# Autodesk Inventor assembly: SAR340 offset 10 mm
(part 2 of 2)
- to_ball1_7_Z@1 <-> to_rail_Z@10 [Mate]: SAR340-40_r:1 ↔ SAR3_ba:7
- to_ball1_7_YZ@1 <-> to_rail_YZ@10 [Angle] (0 deg): SAR340-40_r:1 ↔ SAR3_ba:7
- to_ball1_8_XY@1 <-> to_rail_XY@11 [Mate]: SAR340-40_r:1 ↔ SAR3_ba:8
- to_ball1_8_Z@1 <-> to_rail_Z@11 [Mate]: SAR340-40_r:1 ↔ SAR3_ba:8
- to_ball1_8_YZ@1 <-> to_rail_YZ@11 [Angle] (0 deg): SAR340-40_r:1 ↔ SAR3_ba:8
- to_ball1_9_XY@1 <-> to_rail_XY@12 [Mate]: SAR340-40_r:1 ↔ SAR3_ba:9
- to_ball1_9_Z@1 <-> to_rail_Z@12 [Mate]: SAR340-40_r:1 ↔ SAR3_ba:9
- to_ball1_9_YZ@1 <-> to_rail_YZ@12 [Angle] (0 deg): SAR340-40_r:1 ↔ SAR3_ba:9
- to_ball1_10_XY@1 <-> to_rail_XY@13 [Mate]: SAR340-40_r:1 ↔ SAR3_ba:10
- to_ball1_10_Z@1 <-> to_rail_Z@13 [Mate]: SAR340-40_r:1 ↔ SAR3_ba:10
- to_ball1_10_YZ@1 <-> to_rail_YZ@13 [Angle] (0 deg): SAR340-40_r:1 ↔ SAR3_ba:10
- to_ball1_11_XY@1 <-> to_rail_XY@14 [Mate]: SAR340-40_r:1 ↔ SAR3_ba:11
- to_ball1_11_Z@1 <-> to_rail_Z@14 [Mate]: SAR340-40_r:1 ↔ SAR3_ba:11
- to_ball1_11_YZ@1 <-> to_rail_YZ@14 [Angle] (0 deg): SAR340-40_r:1 ↔ SAR3_ba:11
- to_ball1_12_XY@1 <-> to_rail_XY@15 [Mate]: SAR340-40_r:1 ↔ SAR3_ba:12
- to_ball1_12_Z@1 <-> to_rail_Z@15 [Mate]: SAR340-40_r:1 ↔ SAR3_ba:12
- to_ball1_12_YZ@1 <-> to_rail_YZ@15 [Angle] (0 deg): SAR340-40_r:1 ↔ SAR3_ba:12
- to_ball1_13_XY@1 <-> to_rail_XY@16 [Mate]: SAR340-40_r:1 ↔ SAR3_ba:13
- to_ball1_13_Z@1 <-> to_rail_Z@16 [Mate]: SAR340-40_r:1 ↔ SAR3_ba:13
- to_ball1_13_YZ@1 <-> to_rail_YZ@16 [Angle] (0 deg): SAR340-40_r:1 ↔ SAR3_ba:13
- to_ball1_14_XY@1 <-> to_rail_XY@17 [Mate]: SAR340-40_r:1 ↔ SAR3_ba:14
- to_ball1_14_Z@1 <-> to_rail_Z@17 [Mate]: SAR340-40_r:1 ↔ SAR3_ba:14
- to_ball1_14_YZ@1 <-> to_rail_YZ@17 [Angle] (0 deg): SAR340-40_r:1 ↔ SAR3_ba:14
- to_ball1_15_XY@1 <-> to_rail_XY@18 [Mate]: SAR340-40_r:1 ↔ SAR3_ba:15
- to_ball1_15_Z@1 <-> to_rail_Z@18 [Mate]: SAR340-40_r:1 ↔ SAR3_ba:15
- to_ball1_15_YZ@1 <-> to_rail_YZ@18 [Angle] (0 deg): SAR340-40_r:1 ↔ SAR3_ba:15
- to_ball1_16_XY@1 <-> to_rail_XY@19 [Mate]: SAR340-40_r:1 ↔ SAR3_ba:16
- to_ball1_16_Z@1 <-> to_rail_Z@19 [Mate]: SAR340-40_r:1 ↔ SAR3_ba:16
- to_ball1_16_YZ@1 <-> to_rail_YZ@19 [Angle] (0 deg): SAR340-40_r:1 ↔ SAR3_ba:16
- to_ball1_17_XY@1 <-> to_rail_XY@20 [Mate]: SAR340-40_r:1 ↔ SAR3_ba:17
- to_ball1_17_Z@1 <-> to_rail_Z@20 [Mate]: SAR340-40_r:1 ↔ SAR3_ba:17
- to_ball1_17_YZ@1 <-> to_rail_YZ@20 [Angle] (0 deg): SAR340-40_r:1 ↔ SAR3_ba:17
- to_ball1_18_XY@1 <-> to_rail_XY@21 [Mate]: SAR340-40_r:1 ↔ SAR3_ba:18
- to_ball1_18_Z@1 <-> to_rail_Z@21 [Mate]: SAR340-40_r:1 ↔ SAR3_ba:18
- to_ball1_18_YZ@1 <-> to_rail_YZ@21 [Angle] (0 deg): SAR340-40_r:1 ↔ SAR3_ba:18
- to_ball1_19_XY@1 <-> to_rail_XY@22 [Mate]: SAR340-40_r:1 ↔ SAR3_ba:19
- to_ball1_19_Z@1 <-> to_rail_Z@22 [Mate]: SAR340-40_r:1 ↔ SAR3_ba:19
- to_ball1_19_YZ@1 <-> to_rail_YZ@22 [Angle] (0 deg): SAR340-40_r:1 ↔ SAR3_ba:19
- to_ball1_20_XY@1 <-> to_rail_XY@23 [Mate]: SAR340-40_r:1 ↔ SAR3_ba:20
- to_ball1_20_Z@1 <-> to_rail_Z@23 [Mate]: SAR340-40_r:1 ↔ SAR3_ba:20
- to_ball1_20_YZ@1 <-> to_rail_YZ@23 [Angle] (0 deg): SAR340-40_r:1 ↔ SAR3_ba:20
- to_ball1_21_XY@1 <-> to_rail_XY@24 [Mate]: SAR340-40_r:1 ↔ SAR3_ba:21
- to_ball1_21_Z@1 <-> to_rail_Z@24 [Mate]: SAR340-40_r:1 ↔ SAR3_ba:21
- to_ball1_21_YZ@1 <-> to_rail_YZ@24 [Angle] (0 deg): SAR340-40_r:1 ↔ SAR3_ba:21
- to_ball1_22_XY@1 <-> to_rail_XY@25 [Mate]: SAR340-40_r:1 ↔ SAR3_ba:22
- to_ball1_22_Z@1 <-> to_rail_Z@25 [Mate]: SAR340-40_r:1 ↔ SAR3_ba:22
- to_ball1_22_YZ@1 <-> to_rail_YZ@25 [Angle] (0 deg): SAR340-40_r:1 ↔ SAR3_ba:22
- to_ball1_23_XY@1 <-> to_rail_XY@26 [Mate]: SAR340-40_r:1 ↔ SAR3_ba:23
- to_ball1_23_Z@1 <-> to_rail_Z@26 [Mate]: SAR340-40_r:1 ↔ SAR3_ba:23
- to_ball1_23_YZ@1 <-> to_rail_YZ@26 [Angle] (0 deg): SAR340-40_r:1 ↔ SAR3_ba:23
- to_ball1_24_XY@1 <-> to_rail_XY@27 [Mate]: SAR340-40_r:1 ↔ SAR3_ba:24
- to_ball1_24_Z@1 <-> to_rail_Z@27 [Mate]: SAR340-40_r:1 ↔ SAR3_ba:24
- to_ball1_24_YZ@1 <-> to_rail_YZ@27 [Angle] (0 deg): SAR340-40_r:1 ↔ SAR3_ba:24
- to_ball1_25_XY@1 <-> to_rail_XY@28 [Mate]: SAR340-40_r:1 ↔ SAR3_ba:25
- to_ball1_25_Z@1 <-> to_rail_Z@28 [Mate]: SAR340-40_r:1 ↔ SAR3_ba:25
- to_ball1_25_YZ@1 <-> to_rail_YZ@28 [Angle] (0 deg): SAR340-40_r:1 ↔ SAR3_ba:25
- to_ball1_26_XY@1 <-> to_rail_XY@29 [Mate]: SAR340-40_r:1 ↔ SAR3_ba:26
- to_ball1_26_Z@1 <-> to_rail_Z@29 [Mate]: SAR340-40_r:1 ↔ SAR3_ba:26
- to_ball1_26_YZ@1 <-> to_rail_YZ@29 [Angle] (0 deg): SAR340-40_r:1 ↔ SAR3_ba:26
- to_ball1_27_XY@1 <-> to_rail_XY@30 [Mate]: SAR340-40_r:1 ↔ SAR3_ba:27
- to_ball1_27_Z@1 <-> to_rail_Z@30 [Mate]: SAR340-40_r:1 ↔ SAR3_ba:27
- to_ball1_27_YZ@1 <-> to_rail_YZ@30 [Angle] (0 deg): SAR340-40_r:1 ↔ SAR3_ba:27
- to_ball1_28_XY@1 <-> to_rail_XY@31 [Mate]: SAR340-40_r:1 ↔ SAR3_ba:28
- to_ball1_28_Z@1 <-> to_rail_Z@31 [Mate]: SAR340-40_r:1 ↔ SAR3_ba:28
- to_ball1_28_YZ@1 <-> to_rail_YZ@31 [Angle] (0 deg): SAR340-40_r:1 ↔ SAR3_ba:28
- to_ball1_29_XY@1 <-> to_rail_XY@32 [Mate]: SAR340-40_r:1 ↔ SAR3_ba:29
- to_ball1_29_Z@1 <-> to_rail_Z@32 [Mate]: SAR340-40_r:1 ↔ SAR3_ba:29
- to_ball1_29_YZ@1 <-> to_rail_YZ@32 [Angle] (0 deg): SAR340-40_r:1 ↔ SAR3_ba:29
- to_ball1_30_XY@1 <-> to_rail_XY@33 [Mate]: SAR340-40_r:1 ↔ SAR3_ba:30
- to_ball1_30_Z@1 <-> to_rail_Z@33 [Mate]: SAR340-40_r:1 ↔ SAR3_ba:30
- to_ball1_30_YZ@1 <-> to_rail_YZ@33 [Angle] (0 deg): SAR340-40_r:1 ↔ SAR3_ba:30
- to_ball1_31_XY@1 <-> to_rail_XY@34 [Mate]: SAR340-40_r:1 ↔ SAR3_ba:31
- to_ball1_31_Z@1 <-> to_rail_Z@34 [Mate]: SAR340-40_r:1 ↔ SAR3_ba:31
- to_ball1_31_YZ@1 <-> to_rail_YZ@34 [Angle] (0 deg): SAR340-40_r:1 ↔ SAR3_ba:31
- to_ball1_32_XY@1 <-> to_rail_XY@35 [Mate]: SAR340-40_r:1 ↔ SAR3_ba:32
- to_ball1_32_Z@1 <-> to_rail_Z@35 [Mate]: SAR340-40_r:1 ↔ SAR3_ba:32
- to_ball1_32_YZ@1 <-> to_rail_YZ@35 [Angle] (0 deg): SAR340-40_r:1 ↔ SAR3_ba:32
- to_ball1_33_XY@1 <-> to_rail_XY@36 [Mate]: SAR340-40_r:1 ↔ SAR3_ba:33
- to_ball1_33_Z@1 <-> to_rail_Z@36 [Mate]: SAR340-40_r:1 ↔ SAR3_ba:33
- to_ball1_33_YZ@1 <-> to_rail_YZ@36 [Angle] (0 deg): SAR340-40_r:1 ↔ SAR3_ba:33
- to_ball1_34_XY@1 <-> to_rail_XY@37 [Mate]: SAR340-40_r:1 ↔ SAR3_ba:34
- to_ball1_34_Z@1 <-> to_rail_Z@37 [Mate]: SAR340-40_r:1 ↔ SAR3_ba:34
- to_ball1_34_YZ@1 <-> to_rail_YZ@37 [Angle] (0 deg): SAR340-40_r:1 ↔ SAR3_ba:34
- to_ball1_35_XY@1 <-> to_rail_XY@38 [Mate]: SAR340-40_r:1 ↔ SAR3_ba:35
- to_ball1_35_Z@1 <-> to_rail_Z@38 [Mate]: SAR340-40_r:1 ↔ SAR3_ba:35
- to_ball1_35_YZ@1 <-> to_rail_YZ@38 [Angle] (0 deg): SAR340-40_r:1 ↔ SAR3_ba:35
- to_ball1_36_XY@1 <-> to_rail_XY@39 [Mate]: SAR340-40_r:1 ↔ SAR3_ba:36
- to_ball1_36_Z@1 <-> to_rail_Z@39 [Mate]: SAR340-40_r:1 ↔ SAR3_ba:36
- to_ball1_36_YZ@1 <-> to_rail_YZ@39 [Angle] (0 deg): SAR340-40_r:1 ↔ SAR3_ba:36
- to_ball1_37_XY@1 <-> to_rail_XY@40 [Mate]: SAR340-40_r:1 ↔ SAR3_ba:37
- to_ball1_37_Z@1 <-> to_rail_Z@40 [Mate]: SAR340-40_r:1 ↔ SAR3_ba:37
- to_ball1_37_YZ@1 <-> to_rail_YZ@40 [Angle] (0 deg): SAR340-40_r:1 ↔ SAR3_ba:37
- to_ball2_1_XY@1 <-> to_rail_XY@41 [Mate]: SAR340-40_r:1 ↔ SAR3_ba:38
- to_ball2_1_Z@1 <-> to_rail_Z@41 [Mate]: SAR340-40_r:1 ↔ SAR3_ba:38
- to_ball2_1_YZ@1 <-> to_rail_YZ@41 [Angle] (0 deg): SAR340-40_r:1 ↔ SAR3_ba:38
- to_ball2_2_XY@1 <-> to_rail_XY@42 [Mate]: SAR340-40_r:1 ↔ SAR3_ba:39
- to_ball2_2_Z@1 <-> to_rail_Z@42 [Mate]: SAR340-40_r:1 ↔ SAR3_ba:39
- to_ball2_2_YZ@1 <-> to_rail_YZ@42 [Angle] (0 deg): SAR340-40_r:1 ↔ SAR3_ba:39
- to_ball2_3_XY@1 <-> to_rail_XY@43 [Mate]: SAR340-40_r:1 ↔ SAR3_ba:40
- to_ball2_3_Z@1 <-> to_rail_Z@43 [Mate]: SAR340-40_r:1 ↔ SAR3_ba:40
- to_ball2_3_YZ@1 <-> to_rail_YZ@43 [Angle] (0 deg): SAR340-40_r:1 ↔ SAR3_ba:40
- to_ball2_4_XY@1 <-> to_rail_XY@44 [Mate]: SAR340-40_r:1 ↔ SAR3_ba:41
- to_ball2_4_Z@1 <-> to_rail_Z@44 [Mate]: SAR340-40_r:1 ↔ SAR3_ba:41
- to_ball2_4_YZ@1 <-> to_rail_YZ@44 [Angle] (0 deg): SAR340-40_r:1 ↔ SAR3_ba:41
- to_ball2_5_XY@1 <-> to_rail_XY@45 [Mate]: SAR340-40_r:1 ↔ SAR3_ba:42
- to_ball2_5_Z@1 <-> to_rail_Z@45 [Mate]: SAR340-40_r:1 ↔ SAR3_ba:42
- to_ball2_5_YZ@1 <-> to_rail_YZ@45 [Angle] (0 deg): SAR340-40_r:1 ↔ SAR3_ba:42
- to_ball2_6_XY@1 <-> to_rail_XY@46 [Mate]: SAR340-40_r:1 ↔ SAR3_ba:43
- to_ball2_6_Z@1 <-> to_rail_Z@46 [Mate]: SAR340-40_r:1 ↔ SAR3_ba:43
- to_ball2_6_YZ@1 <-> to_rail_YZ@46 [Angle] (0 deg): SAR340-40_r:1 ↔ SAR3_ba:43
- to_ball2_7_XY@1 <-> to_rail_XY@47 [Mate]: SAR340-40_r:1 ↔ SAR3_ba:44
- to_ball2_7_Z@1 <-> to_rail_Z@47 [Mate]: SAR340-40_r:1 ↔ SAR3_ba:44
- to_ball2_7_YZ@1 <-> to_rail_YZ@47 [Angle] (0 deg): SAR340-40_r:1 ↔ SAR3_ba:44
- to_ball2_8_XY@1 <-> to_rail_XY@48 [Mate]: SAR340-40_r:1 ↔ SAR3_ba:45
- to_ball2_8_Z@1 <-> to_rail_Z@48 [Mate]: SAR340-40_r:1 ↔ SAR3_ba:45
- to_ball2_8_YZ@1 <-> to_rail_YZ@48 [Angle] (0 deg): SAR340-40_r:1 ↔ SAR3_ba:45
- to_ball2_9_XY@1 <-> to_rail_XY@49 [Mate]: SAR340-40_r:1 ↔ SAR3_ba:46
- to_ball2_9_Z@1 <-> to_rail_Z@49 [Mate]: SAR340-40_r:1 ↔ SAR3_ba:46
- to_ball2_9_YZ@1 <-> to_rail_YZ@49 [Angle] (0 deg): SAR340-40_r:1 ↔ SAR3_ba:46
- to_ball2_10_XY@1 <-> to_rail_XY@50 [Mate]: SAR340-40_r:1 ↔ SAR3_ba:47
- to_ball2_10_Z@1 <-> to_rail_Z@50 [Mate]: SAR340-40_r:1 ↔ SAR3_ba:47
- to_ball2_10_YZ@1 <-> to_rail_YZ@50 [Angle] (0 deg): SAR340-40_r:1 ↔ SAR3_ba:47
- to_ball2_11_XY@1 <-> to_rail_XY@51 [Mate]: SAR340-40_r:1 ↔ SAR3_ba:48
- to_ball2_11_Z@1 <-> to_rail_Z@51 [Mate]: SAR340-40_r:1 ↔ SAR3_ba:48
- to_ball2_11_YZ@1 <-> to_rail_YZ@51 [Angle] (0 deg): SAR340-40_r:1 ↔ SAR3_ba:48
- to_ball2_12_XY@1 <-> to_rail_XY@52 [Mate]: SAR340-40_r:1 ↔ SAR3_ba:49
- to_ball2_12_Z@1 <-> to_rail_Z@52 [Mate]: SAR340-40_r:1 ↔ SAR3_ba:49
- to_ball2_12_YZ@1 <-> to_rail_YZ@52 [Angle] (0 deg): SAR340-40_r:1 ↔ SAR3_ba:49
- to_ball2_13_XY@1 <-> to_rail_XY@53 [Mate]: SAR340-40_r:1 ↔ SAR3_ba:50
- to_ball2_13_Z@1 <-> to_rail_Z@53 [Mate]: SAR340-40_r:1 ↔ SAR3_ba:50
- to_ball2_13_YZ@1 <-> to_rail_YZ@53 [Angle] (0 deg): SAR340-40_r:1 ↔ SAR3_ba:50
- to_ball2_14_XY@1 <-> to_rail_XY@54 [Mate]: SAR340-40_r:1 ↔ SAR3_ba:51
- to_ball2_14_Z@1 <-> to_rail_Z@54 [Mate]: SAR340-40_r:1 ↔ SAR3_ba:51
- to_ball2_14_YZ@1 <-> to_rail_YZ@54 [Angle] (0 deg): SAR340-40_r:1 ↔ SAR3_ba:51
- to_ball2_15_XY@1 <-> to_rail_XY@55 [Mate]: SAR340-40_r:1 ↔ SAR3_ba:52
- to_ball2_15_Z@1 <-> to_rail_Z@55 [Mate]: SAR340-40_r:1 ↔ SAR3_ba:52
- to_ball2_15_YZ@1 <-> to_rail_YZ@55 [Angle] (0 deg): SAR340-40_r:1 ↔ SAR3_ba:52
- to_ball2_16_XY@1 <-> to_rail_XY@56 [Mate]: SAR340-40_r:1 ↔ SAR3_ba:53
- to_ball2_16_Z@1 <-> to_rail_Z@56 [Mate]: SAR340-40_r:1 ↔ SAR3_ba:53
- to_ball2_16_YZ@1 <-> to_rail_YZ@56 [Angle] (0 deg): SAR340-40_r:1 ↔ SAR3_ba:53
- to_ball2_17_XY@1 <-> to_rail_XY@57 [Mate]: SAR340-40_r:1 ↔ SAR3_ba:54
- to_ball2_17_Z@1 <-> to_rail_Z@57 [Mate]: SAR340-40_r:1 ↔ SAR3_ba:54
- to_ball2_17_YZ@1 <-> to_rail_YZ@57 [Angle] (0 deg): SAR340-40_r:1 ↔ SAR3_ba:54
- to_ball2_18_XY@1 <-> to_rail_XY@58 [Mate]: SAR340-40_r:1 ↔ SAR3_ba:55
- to_ball2_18_Z@1 <-> to_rail_Z@58 [Mate]: SAR340-40_r:1 ↔ SAR3_ba:55
- to_ball2_18_YZ@1 <-> to_rail_YZ@58 [Angle] (0 deg): SAR340-40_r:1 ↔ SAR3_ba:55
- to_ball2_19_XY@1 <-> to_rail_XY@59 [Mate]: SAR340-40_r:1 ↔ SAR3_ba:56
- to_ball2_19_Z@1 <-> to_rail_Z@59 [Mate]: SAR340-40_r:1 ↔ SAR3_ba:56
- to_ball2_19_YZ@1 <-> to_rail_YZ@59 [Angle] (0 deg): SAR340-40_r:1 ↔ SAR3_ba:56
- to_ball2_20_XY@1 <-> to_rail_XY@60 [Mate]: SAR340-40_r:1 ↔ SAR3_ba:57
- to_ball2_20_Z@1 <-> to_rail_Z@60 [Mate]: SAR340-40_r:1 ↔ SAR3_ba:57
- to_ball2_20_YZ@1 <-> to_rail_YZ@60 [Angle] (0 deg): SAR340-40_r:1 ↔ SAR3_ba:57
- to_ball2_21_XY@1 <-> to_rail_XY@61 [Mate]: SAR340-40_r:1 ↔ SAR3_ba:58
- to_ball2_21_Z@1 <-> to_rail_Z@61 [Mate]: SAR340-40_r:1 ↔ SAR3_ba:58
- to_ball2_21_YZ@1 <-> to_rail_YZ@61 [Angle] (0 deg): SAR340-40_r:1 ↔ SAR3_ba:58
- to_ball2_22_XY@1 <-> to_rail_XY@62 [Mate]: SAR340-40_r:1 ↔ SAR3_ba:59
- to_ball2_22_Z@1 <-> to_rail_Z@62 [Mate]: SAR340-40_r:1 ↔ SAR3_ba:59
- to_ball2_22_YZ@1 <-> to_rail_YZ@62 [Angle] (0 deg): SAR340-40_r:1 ↔ SAR3_ba:59
- to_ball2_23_XY@1 <-> to_rail_XY@63 [Mate]: SAR340-40_r:1 ↔ SAR3_ba:60
- to_ball2_23_Z@1 <-> to_rail_Z@63 [Mate]: SAR340-40_r:1 ↔ SAR3_ba:60
- to_ball2_23_YZ@1 <-> to_rail_YZ@63 [Angle] (0 deg): SAR340-40_r:1 ↔ SAR3_ba:60
- to_ball2_24_XY@1 <-> to_rail_XY@64 [Mate]: SAR340-40_r:1 ↔ SAR3_ba:61
- to_ball2_24_Z@1 <-> to_rail_Z@64 [Mate]: SAR340-40_r:1 ↔ SAR3_ba:61
- to_ball2_24_YZ@1 <-> to_rail_YZ@64 [Angle] (0 deg): SAR340-40_r:1 ↔ SAR3_ba:61
- to_ball2_25_XY@1 <-> to_rail_XY@65 [Mate]: SAR340-40_r:1 ↔ SAR3_ba:62
- to_ball2_25_Z@1 <-> to_rail_Z@65 [Mate]: SAR340-40_r:1 ↔ SAR3_ba:62
- to_ball2_25_YZ@1 <-> to_rail_YZ@65 [Angle] (0 deg): SAR340-40_r:1 ↔ SAR3_ba:62
- to_ball2_26_XY@1 <-> to_rail_XY@66 [Mate]: SAR340-40_r:1 ↔ SAR3_ba:63
- to_ball2_26_Z@1 <-> to_rail_Z@66 [Mate]: SAR340-40_r:1 ↔ SAR3_ba:63
- to_ball2_26_YZ@1 <-> to_rail_YZ@66 [Angle] (0 deg): SAR340-40_r:1 ↔ SAR3_ba:63
- to_ball2_27_XY@1 <-> to_rail_XY@67 [Mate]: SAR340-40_r:1 ↔ SAR3_ba:64
- to_ball2_27_Z@1 <-> to_rail_Z@67 [Mate]: SAR340-40_r:1 ↔ SAR3_ba:64
- to_ball2_27_YZ@1 <-> to_rail_YZ@67 [Angle] (0 deg): SAR340-40_r:1 ↔ SAR3_ba:64
- to_ball2_28_XY@1 <-> to_rail_XY@68 [Mate]: SAR340-40_r:1 ↔ SAR3_ba:65
- to_ball2_28_Z@1 <-> to_rail_Z@68 [Mate]: SAR340-40_r:1 ↔ SAR3_ba:65
- to_ball2_28_YZ@1 <-> to_rail_YZ@68 [Angle] (0 deg): SAR340-40_r:1 ↔ SAR3_ba:65
- to_ball2_29_XY@1 <-> to_rail_XY@69 [Mate]: SAR340-40_r:1 ↔ SAR3_ba:66
- to_ball2_29_Z@1 <-> to_rail_Z@69 [Mate]: SAR340-40_r:1 ↔ SAR3_ba:66
- to_ball2_29_YZ@1 <-> to_rail_YZ@69 [Angle] (0 deg): SAR340-40_r:1 ↔ SAR3_ba:66
- to_ball2_30_XY@1 <-> to_rail_XY@70 [Mate]: SAR340-40_r:1 ↔ SAR3_ba:67
- to_ball2_30_Z@1 <-> to_rail_Z@70 [Mate]: SAR340-40_r:1 ↔ SAR3_ba:67
- to_ball2_30_YZ@1 <-> to_rail_YZ@70 [Angle] (0 deg): SAR340-40_r:1 ↔ SAR3_ba:67
- to_ball2_31_XY@1 <-> to_rail_XY@71 [Mate]: SAR340-40_r:1 ↔ SAR3_ba:68
- to_ball2_31_Z@1 <-> to_rail_Z@71 [Mate]: SAR340-40_r:1 ↔ SAR3_ba:68
- to_ball2_31_YZ@1 <-> to_rail_YZ@71 [Angle] (0 deg): SAR340-40_r:1 ↔ SAR3_ba:68
- to_ball2_32_XY@1 <-> to_rail_XY@72 [Mate]: SAR340-40_r:1 ↔ SAR3_ba:69
- to_ball2_32_Z@1 <-> to_rail_Z@72 [Mate]: SAR340-40_r:1 ↔ SAR3_ba:69
- to_ball2_32_YZ@1 <-> to_rail_YZ@72 [Angle] (0 deg): SAR340-40_r:1 ↔ SAR3_ba:69
- to_ball2_33_XY@1 <-> to_rail_XY@73 [Mate]: SAR340-40_r:1 ↔ SAR3_ba:70
- to_ball2_33_Z@1 <-> to_rail_Z@73 [Mate]: SAR340-40_r:1 ↔ SAR3_ba:70
- to_ball2_33_YZ@1 <-> to_rail_YZ@73 [Angle] (0 deg): SAR340-40_r:1 ↔ SAR3_ba:70
- to_ball2_34_XY@1 <-> to_rail_XY@74 [Mate]: SAR340-40_r:1 ↔ SAR3_ba:71
- to_ball2_34_Z@1 <-> to_rail_Z@74 [Mate]: SAR340-40_r:1 ↔ SAR3_ba:71
- to_ball2_34_YZ@1 <-> to_rail_YZ@74 [Angle] (0 deg): SAR340-40_r:1 ↔ SAR3_ba:71
- to_ball2_35_XY@1 <-> to_rail_XY@75 [Mate]: SAR340-40_r:1 ↔ SAR3_ba:72
- to_ball2_35_Z@1 <-> to_rail_Z@75 [Mate]: SAR340-40_r:1 ↔ SAR3_ba:72
- to_ball2_35_YZ@1 <-> to_rail_YZ@75 [Angle] (0 deg): SAR340-40_r:1 ↔ SAR3_ba:72
- to_ball2_36_XY@1 <-> to_rail_XY@76 [Mate]: SAR340-40_r:1 ↔ SAR3_ba:73
- to_ball2_36_Z@1 <-> to_rail_Z@76 [Mate]: SAR340-40_r:1 ↔ SAR3_ba:73
- to_ball2_36_YZ@1 <-> to_rail_YZ@76 [Angle] (0 deg): SAR340-40_r:1 ↔ SAR3_ba:73
- to_ball2_37_XY@1 <-> to_rail_XY@77 [Mate]: SAR340-40_r:1 ↔ SAR3_ba:74
- to_ball2_37_Z@1 <-> to_rail_Z@77 [Mate]: SAR340-40_r:1 ↔ SAR3_ba:74
- to_ball2_37_YZ@1 <-> to_rail_YZ@77 [Angle] (0 deg): SAR340-40_r:1 ↔ SAR3_ba:74
- to_ball3_1_XY@1 <-> to_rail_XY@78 [Mate]: SAR340-40_r:1 ↔ SAR3_ba:75
- to_ball3_1_Z@1 <-> to_rail_Z@78 [Mate]: SAR340-40_r:1 ↔ SAR3_ba:75
- to_ball3_1_YZ@1 <-> to_rail_YZ@78 [Angle] (0 deg): SAR340-40_r:1 ↔ SAR3_ba:75
- to_ball3_2_XY@1 <-> to_rail_XY@79 [Mate]: SAR340-40_r:1 ↔ SAR3_ba:76
- to_ball3_2_Z@1 <-> to_rail_Z@79 [Mate]: SAR340-40_r:1 ↔ SAR3_ba:76
- to_ball3_2_YZ@1 <-> to_rail_YZ@79 [Angle] (0 deg): SAR340-40_r:1 ↔ SAR3_ba:76
- to_ball3_3_XY@1 <-> to_rail_XY@80 [Mate]: SAR340-40_r:1 ↔ SAR3_ba:77
- to_ball3_3_Z@1 <-> to_rail_Z@80 [Mate]: SAR340-40_r:1 ↔ SAR3_ba:77
- to_ball3_3_YZ@1 <-> to_rail_YZ@80 [Angle] (0 deg): SAR340-40_r:1 ↔ SAR3_ba:77
- to_ball3_4_XY@1 <-> to_rail_XY@81 [Mate]: SAR340-40_r:1 ↔ SAR3_ba:78
- to_ball3_4_Z@1 <-> to_rail_Z@81 [Mate]: SAR340-40_r:1 ↔ SAR3_ba:78
- to_ball3_4_YZ@1 <-> to_rail_YZ@81 [Angle] (0 deg): SAR340-40_r:1 ↔ SAR3_ba:78
- to_ball3_5_XY@1 <-> to_rail_XY@82 [Mate]: SAR340-40_r:1 ↔ SAR3_ba:79
- to_ball3_5_Z@1 <-> to_rail_Z@82 [Mate]: SAR340-40_r:1 ↔ SAR3_ba:79
- to_ball3_5_YZ@1 <-> to_rail_YZ@82 [Angle] (0 deg): SAR340-40_r:1 ↔ SAR3_ba:79
- to_ball3_6_XY@1 <-> to_rail_XY@83 [Mate]: SAR340-40_r:1 ↔ SAR3_ba:80
- to_ball3_6_Z@1 <-> to_rail_Z@83 [Mate]: SAR340-40_r:1 ↔ SAR3_ba:80
- to_ball3_6_YZ@1 <-> to_rail_YZ@83 [Angle] (0 deg): SAR340-40_r:1 ↔ SAR3_ba:80
- to_ball3_7_XY@1 <-> to_rail_XY@84 [Mate]: SAR340-40_r:1 ↔ SAR3_ba:81
- to_ball3_7_Z@1 <-> to_rail_Z@84 [Mate]: SAR340-40_r:1 ↔ SAR3_ba:81
- to_ball3_7_YZ@1 <-> to_rail_YZ@84 [Angle] (0 deg): SAR340-40_r:1 ↔ SAR3_ba:81
- to_ball3_8_XY@1 <-> to_rail_XY@85 [Mate]: SAR340-40_r:1 ↔ SAR3_ba:82
- to_ball3_8_Z@1 <-> to_rail_Z@85 [Mate]: SAR340-40_r:1 ↔ SAR3_ba:82
- to_ball3_8_YZ@1 <-> to_rail_YZ@85 [Angle] (0 deg): SAR340-40_r:1 ↔ SAR3_ba:82
- to_ball3_9_XY@1 <-> to_rail_XY@86 [Mate]: SAR340-40_r:1 ↔ SAR3_ba:83
- to_ball3_9_Z@1 <-> to_rail_Z@86 [Mate]: SAR340-40_r:1 ↔ SAR3_ba:83
- to_ball3_9_YZ@1 <-> to_rail_YZ@86 [Angle] (0 deg): SAR340-40_r:1 ↔ SAR3_ba:83
- to_ball3_10_XY@1 <-> to_rail_XY@87 [Mate]: SAR340-40_r:1 ↔ SAR3_ba:84
- to_ball3_10_Z@1 <-> to_rail_Z@87 [Mate]: SAR340-40_r:1 ↔ SAR3_ba:84
- to_ball3_10_YZ@1 <-> to_rail_YZ@87 [Angle] (0 deg): SAR340-40_r:1 ↔ SAR3_ba:84
- to_ball3_11_XY@1 <-> to_rail_XY@88 [Mate]: SAR340-40_r:1 ↔ SAR3_ba:85
- to_ball3_11_Z@1 <-> to_rail_Z@88 [Mate]: SAR340-40_r:1 ↔ SAR3_ba:85
- to_ball3_11_YZ@1 <-> to_rail_YZ@88 [Angle] (0 deg): SAR340-40_r:1 ↔ SAR3_ba:85
- to_ball3_12_XY@1 <-> to_rail_XY@89 [Mate]: SAR340-40_r:1 ↔ SAR3_ba:86
- to_ball3_12_Z@1 <-> to_rail_Z@89 [Mate]: SAR340-40_r:1 ↔ SAR3_ba:86
- to_ball3_12_YZ@1 <-> to_rail_YZ@89 [Angle] (0 deg): SAR340-40_r:1 ↔ SAR3_ba:86
- to_ball3_13_XY@1 <-> to_rail_XY@90 [Mate]: SAR340-40_r:1 ↔ SAR3_ba:87
- to_ball3_13_Z@1 <-> to_rail_Z@90 [Mate]: SAR340-40_r:1 ↔ SAR3_ba:87
- to_ball3_13_YZ@1 <-> to_rail_YZ@90 [Angle] (0 deg): SAR340-40_r:1 ↔ SAR3_ba:87
- to_ball3_14_XY@1 <-> to_rail_XY@91 [Mate]: SAR340-40_r:1 ↔ SAR3_ba:88
- to_ball3_14_Z@1 <-> to_rail_Z@91 [Mate]: SAR340-40_r:1 ↔ SAR3_ba:88
- to_ball3_14_YZ@1 <-> to_rail_YZ@91 [Angle] (0 deg): SAR340-40_r:1 ↔ SAR3_ba:88
- to_ball3_15_XY@1 <-> to_rail_XY@92 [Mate]: SAR340-40_r:1 ↔ SAR3_ba:89
- to_ball3_15_Z@1 <-> to_rail_Z@92 [Mate]: SAR340-40_r:1 ↔ SAR3_ba:89
- to_ball3_15_YZ@1 <-> to_rail_YZ@92 [Angle] (0 deg): SAR340-40_r:1 ↔ SAR3_ba:89
- to_ball3_16_XY@1 <-> to_rail_XY@93 [Mate]: SAR340-40_r:1 ↔ SAR3_ba:90
- to_ball3_16_Z@1 <-> to_rail_Z@93 [Mate]: SAR340-40_r:1 ↔ SAR3_ba:90
- to_ball3_16_YZ@1 <-> to_rail_YZ@93 [Angle] (0 deg): SAR340-40_r:1 ↔ SAR3_ba:90
- to_ball3_17_XY@1 <-> to_rail_XY@94 [Mate]: SAR340-40_r:1 ↔ SAR3_ba:91
- to_ball3_17_Z@1 <-> to_rail_Z@94 [Mate]: SAR340-40_r:1 ↔ SAR3_ba:91
- to_ball3_17_YZ@1 <-> to_rail_YZ@94 [Angle] (0 deg): SAR340-40_r:1 ↔ SAR3_ba:91
- to_ball3_18_XY@1 <-> to_rail_XY@95 [Mate]: SAR340-40_r:1 ↔ SAR3_ba:92
- to_ball3_18_Z@1 <-> to_rail_Z@95 [Mate]: SAR340-40_r:1 ↔ SAR3_ba:92
- to_ball3_18_YZ@1 <-> to_rail_YZ@95 [Angle] (0 deg): SAR340-40_r:1 ↔ SAR3_ba:92
- to_ball3_19_XY@1 <-> to_rail_XY@96 [Mate]: SAR340-40_r:1 ↔ SAR3_ba:93
- to_ball3_19_Z@1 <-> to_rail_Z@96 [Mate]: SAR340-40_r:1 ↔ SAR3_ba:93
- to_ball3_19_YZ@1 <-> to_rail_YZ@96 [Angle] (0 deg): SAR340-40_r:1 ↔ SAR3_ba:93
- to_ball3_20_XY@1 <-> to_rail_XY@97 [Mate]: SAR340-40_r:1 ↔ SAR3_ba:94
- to_ball3_20_Z@1 <-> to_rail_Z@97 [Mate]: SAR340-40_r:1 ↔ SAR3_ba:94
- to_ball3_20_YZ@1 <-> to_rail_YZ@97 [Angle] (0 deg): SAR340-40_r:1 ↔ SAR3_ba:94
- to_ball3_21_XY@1 <-> to_rail_XY@98 [Mate]: SAR340-40_r:1 ↔ SAR3_ba:95
- to_ball3_21_Z@1 <-> to_rail_Z@98 [Mate]: SAR340-40_r:1 ↔ SAR3_ba:95
- to_ball3_21_YZ@1 <-> to_rail_YZ@98 [Angle] (0 deg): SAR340-40_r:1 ↔ SAR3_ba:95
- to_ball3_22_XY@1 <-> to_rail_XY@99 [Mate]: SAR340-40_r:1 ↔ SAR3_ba:96
- to_ball3_22_Z@1 <-> to_rail_Z@99 [Mate]: SAR340-40_r:1 ↔ SAR3_ba:96
- to_ball3_22_YZ@1 <-> to_rail_YZ@99 [Angle] (0 deg): SAR340-40_r:1 ↔ SAR3_ba:96
- to_ball3_23_XY@1 <-> to_rail_XY@100 [Mate]: SAR340-40_r:1 ↔ SAR3_ba:97
- to_ball3_23_Z@1 <-> to_rail_Z@100 [Mate]: SAR340-40_r:1 ↔ SAR3_ba:97
- to_ball3_23_YZ@1 <-> to_rail_YZ@100 [Angle] (0 deg): SAR340-40_r:1 ↔ SAR3_ba:97
- to_ball3_24_XY@1 <-> to_rail_XY@101 [Mate]: SAR340-40_r:1 ↔ SAR3_ba:98
- to_ball3_24_Z@1 <-> to_rail_Z@101 [Mate]: SAR340-40_r:1 ↔ SAR3_ba:98
- to_ball3_24_YZ@1 <-> to_rail_YZ@101 [Angle] (0 deg): SAR340-40_r:1 ↔ SAR3_ba:98
- to_ball3_25_XY@1 <-> to_rail_XY@102 [Mate]: SAR340-40_r:1 ↔ SAR3_ba:99
- to_ball3_25_Z@1 <-> to_rail_Z@102 [Mate]: SAR340-40_r:1 ↔ SAR3_ba:99
- to_ball3_25_YZ@1 <-> to_rail_YZ@102 [Angle] (0 deg): SAR340-40_r:1 ↔ SAR3_ba:99
- to_ball3_26_XY@1 <-> to_rail_XY@103 [Mate]: SAR340-40_r:1 ↔ SAR3_ba:100
- to_ball3_26_Z@1 <-> to_rail_Z@103 [Mate]: SAR340-40_r:1 ↔ SAR3_ba:100
- to_ball3_26_YZ@1 <-> to_rail_YZ@103 [Angle] (0 deg): SAR340-40_r:1 ↔ SAR3_ba:100
- to_ball3_27_XY@1 <-> to_rail_XY@104 [Mate]: SAR340-40_r:1 ↔ SAR3_ba:101
- to_ball3_27_Z@1 <-> to_rail_Z@104 [Mate]: SAR340-40_r:1 ↔ SAR3_ba:101
- to_ball3_27_YZ@1 <-> to_rail_YZ@104 [Angle] (0 deg): SAR340-40_r:1 ↔ SAR3_ba:101
- to_ball3_28_XY@1 <-> to_rail_XY@105 [Mate]: SAR340-40_r:1 ↔ SAR3_ba:102
- to_ball3_28_Z@1 <-> to_rail_Z@105 [Mate]: SAR340-40_r:1 ↔ SAR3_ba:102
- to_ball3_28_YZ@1 <-> to_rail_YZ@105 [Angle] (0 deg): SAR340-40_r:1 ↔ SAR3_ba:102
- to_ball3_29_XY@1 <-> to_rail_XY@106 [Mate]: SAR340-40_r:1 ↔ SAR3_ba:103
- to_ball3_29_Z@1 <-> to_rail_Z@106 [Mate]: SAR340-40_r:1 ↔ SAR3_ba:103
- to_ball3_29_YZ@1 <-> to_rail_YZ@106 [Angle] (0 deg): SAR340-40_r:1 ↔ SAR3_ba:103
- to_ball3_30_XY@1 <-> to_rail_XY@107 [Mate]: SAR340-40_r:1 ↔ SAR3_ba:104
- to_ball3_30_Z@1 <-> to_rail_Z@107 [Mate]: SAR340-40_r:1 ↔ SAR3_ba:104
- to_ball3_30_YZ@1 <-> to_rail_YZ@107 [Angle] (0 deg): SAR340-40_r:1 ↔ SAR3_ba:104
- to_ball3_31_XY@1 <-> to_rail_XY@108 [Mate]: SAR340-40_r:1 ↔ SAR3_ba:105
- to_ball3_31_Z@1 <-> to_rail_Z@108 [Mate]: SAR340-40_r:1 ↔ SAR3_ba:105
- to_ball3_31_YZ@1 <-> to_rail_YZ@108 [Angle] (0 deg): SAR340-40_r:1 ↔ SAR3_ba:105
- to_ball3_32_XY@1 <-> to_rail_XY@109 [Mate]: SAR340-40_r:1 ↔ SAR3_ba:106
- to_ball3_32_Z@1 <-> to_rail_Z@109 [Mate]: SAR340-40_r:1 ↔ SAR3_ba:106
- to_ball3_32_YZ@1 <-> to_rail_YZ@109 [Angle] (0 deg): SAR340-40_r:1 ↔ SAR3_ba:106
- to_ball3_33_XY@1 <-> to_rail_XY@110 [Mate]: SAR340-40_r:1 ↔ SAR3_ba:107
- to_ball3_33_Z@1 <-> to_rail_Z@110 [Mate]: SAR340-40_r:1 ↔ SAR3_ba:107
- to_ball3_33_YZ@1 <-> to_rail_YZ@110 [Angle] (0 deg): SAR340-40_r:1 ↔ SAR3_ba:107
- to_ball3_34_XY@1 <-> to_rail_XY@111 [Mate]: SAR340-40_r:1 ↔ SAR3_ba:108
- to_ball3_34_Z@1 <-> to_rail_Z@111 [Mate]: SAR340-40_r:1 ↔ SAR3_ba:108
- to_ball3_34_YZ@1 <-> to_rail_YZ@111 [Angle] (0 deg): SAR340-40_r:1 ↔ SAR3_ba:108
- to_ball3_35_XY@1 <-> to_rail_XY@112 [Mate]: SAR340-40_r:1 ↔ SAR3_ba:109
- to_ball3_35_Z@1 <-> to_rail_Z@112 [Mate]: SAR340-40_r:1 ↔ SAR3_ba:109
- to_ball3_35_YZ@1 <-> to_rail_YZ@112 [Angle] (0 deg): SAR340-40_r:1 ↔ SAR3_ba:109
- to_ball3_36_XY@1 <-> to_rail_XY@113 [Mate]: SAR340-40_r:1 ↔ SAR3_ba:110
- to_ball3_36_Z@1 <-> to_rail_Z@113 [Mate]: SAR340-40_r:1 ↔ SAR3_ba:110
- to_ball3_36_YZ@1 <-> to_rail_YZ@113 [Angle] (0 deg): SAR340-40_r:1 ↔ SAR3_ba:110
- to_ball3_37_XY@1 <-> to_rail_XY@114 [Mate]: SAR340-40_r:1 ↔ SAR3_ba:111
- to_ball3_37_Z@1 <-> to_rail_Z@114 [Mate]: SAR340-40_r:1 ↔ SAR3_ba:111
- to_ball3_37_YZ@1 <-> to_rail_YZ@114 [Angle] (0 deg): SAR340-40_r:1 ↔ SAR3_ba:111
- to_ball4_1_XY@1 <-> to_rail_XY@115 [Mate]: SAR340-40_r:1 ↔ SAR3_ba:112
- to_ball4_1_Z@1 <-> to_rail_Z@115 [Mate]: SAR340-40_r:1 ↔ SAR3_ba:112
- to_ball4_1_YZ@1 <-> to_rail_YZ@115 [Angle] (0 deg): SAR340-40_r:1 ↔ SAR3_ba:112
- to_ball4_2_XY@1 <-> to_rail_XY@116 [Mate]: SAR340-40_r:1 ↔ SAR3_ba:113
- to_ball4_2_Z@1 <-> to_rail_Z@116 [Mate]: SAR340-40_r:1 ↔ SAR3_ba:113
- to_ball4_2_YZ@1 <-> to_rail_YZ@116 [Angle] (0 deg): SAR340-40_r:1 ↔ SAR3_ba:113
- to_ball4_3_XY@1 <-> to_rail_XY@117 [Mate]: SAR340-40_r:1 ↔ SAR3_ba:114
- to_ball4_3_Z@1 <-> to_rail_Z@117 [Mate]: SAR340-40_r:1 ↔ SAR3_ba:114
- to_ball4_3_YZ@1 <-> to_rail_YZ@117 [Angle] (0 deg): SAR340-40_r:1 ↔ SAR3_ba:114
- to_ball4_4_XY@1 <-> to_rail_XY@118 [Mate]: SAR340-40_r:1 ↔ SAR3_ba:115
- to_ball4_4_Z@1 <-> to_rail_Z@118 [Mate]: SAR340-40_r:1 ↔ SAR3_ba:115
- to_ball4_4_YZ@1 <-> to_rail_YZ@118 [Angle] (0 deg): SAR340-40_r:1 ↔ SAR3_ba:115
- to_ball4_5_XY@1 <-> to_rail_XY@119 [Mate]: SAR340-40_r:1 ↔ SAR3_ba:116
- to_ball4_5_Z@1 <-> to_rail_Z@119 [Mate]: SAR340-40_r:1 ↔ SAR3_ba:116
- to_ball4_5_YZ@1 <-> to_rail_YZ@119 [Angle] (0 deg): SAR340-40_r:1 ↔ SAR3_ba:116
- to_ball4_6_XY@1 <-> to_rail_XY@120 [Mate]: SAR340-40_r:1 ↔ SAR3_ba:117
- to_ball4_6_Z@1 <-> to_rail_Z@120 [Mate]: SAR340-40_r:1 ↔ SAR3_ba:117
- to_ball4_6_YZ@1 <-> to_rail_YZ@120 [Angle] (0 deg): SAR340-40_r:1 ↔ SAR3_ba:117
- to_ball4_7_XY@1 <-> to_rail_XY@121 [Mate]: SAR340-40_r:1 ↔ SAR3_ba:118
- to_ball4_7_Z@1 <-> to_rail_Z@121 [Mate]: SAR340-40_r:1 ↔ SAR3_ba:118
- to_ball4_7_YZ@1 <-> to_rail_YZ@121 [Angle] (0 deg): SAR340-40_r:1 ↔ SAR3_ba:118
- to_ball4_8_XY@1 <-> to_rail_XY@122 [Mate]: SAR340-40_r:1 ↔ SAR3_ba:119
- to_ball4_8_Z@1 <-> to_rail_Z@122 [Mate]: SAR340-40_r:1 ↔ SAR3_ba:119
- to_ball4_8_YZ@1 <-> to_rail_YZ@122 [Angle] (0 deg): SAR340-40_r:1 ↔ SAR3_ba:119
- to_ball4_9_XY@1 <-> to_rail_XY@123 [Mate]: SAR340-40_r:1 ↔ SAR3_ba:120
- to_ball4_9_Z@1 <-> to_rail_Z@123 [Mate]: SAR340-40_r:1 ↔ SAR3_ba:120
- to_ball4_9_YZ@1 <-> to_rail_YZ@123 [Angle] (0 deg): SAR340-40_r:1 ↔ SAR3_ba:120
- to_ball4_10_XY@1 <-> to_rail_XY@124 [Mate]: SAR340-40_r:1 ↔ SAR3_ba:121
- to_ball4_10_Z@1 <-> to_rail_Z@124 [Mate]: SAR340-40_r:1 ↔ SAR3_ba:121
- to_ball4_10_YZ@1 <-> to_rail_YZ@124 [Angle] (0 deg): SAR340-40_r:1 ↔ SAR3_ba:121
- to_ball4_11_XY@1 <-> to_rail_XY@125 [Mate]: SAR340-40_r:1 ↔ SAR3_ba:122
- to_ball4_11_Z@1 <-> to_rail_Z@125 [Mate]: SAR340-40_r:1 ↔ SAR3_ba:122
- to_ball4_11_YZ@1 <-> to_rail_YZ@125 [Angle] (0 deg): SAR340-40_r:1 ↔ SAR3_ba:122
- to_ball4_12_XY@1 <-> to_rail_XY@126 [Mate]: SAR340-40_r:1 ↔ SAR3_ba:123
- to_ball4_12_Z@1 <-> to_rail_Z@126 [Mate]: SAR340-40_r:1 ↔ SAR3_ba:123
- to_ball4_12_YZ@1 <-> to_rail_YZ@126 [Angle] (0 deg): SAR340-40_r:1 ↔ SAR3_ba:123
- to_ball4_13_XY@1 <-> to_rail_XY@127 [Mate]: SAR340-40_r:1 ↔ SAR3_ba:124
- to_ball4_13_Z@1 <-> to_rail_Z@127 [Mate]: SAR340-40_r:1 ↔ SAR3_ba:124
- to_ball4_13_YZ@1 <-> to_rail_YZ@127 [Angle] (0 deg): SAR340-40_r:1 ↔ SAR3_ba:124
- to_ball4_14_XY@1 <-> to_rail_XY@128 [Mate]: SAR340-40_r:1 ↔ SAR3_ba:125
- to_ball4_14_Z@1 <-> to_rail_Z@128 [Mate]: SAR340-40_r:1 ↔ SAR3_ba:125
- to_ball4_14_YZ@1 <-> to_rail_YZ@128 [Angle] (0 deg): SAR340-40_r:1 ↔ SAR3_ba:125
- to_ball4_15_XY@1 <-> to_rail_XY@129 [Mate]: SAR340-40_r:1 ↔ SAR3_ba:126
- to_ball4_15_Z@1 <-> to_rail_Z@129 [Mate]: SAR340-40_r:1 ↔ SAR3_ba:126
- to_ball4_15_YZ@1 <-> to_rail_YZ@129 [Angle] (0 deg): SAR340-40_r:1 ↔ SAR3_ba:126
- to_ball4_16_XY@1 <-> to_rail_XY@130 [Mate]: SAR340-40_r:1 ↔ SAR3_ba:127
- to_ball4_16_Z@1 <-> to_rail_Z@130 [Mate]: SAR340-40_r:1 ↔ SAR3_ba:127
- to_ball4_16_YZ@1 <-> to_rail_YZ@130 [Angle] (0 deg): SAR340-40_r:1 ↔ SAR3_ba:127
- to_ball4_17_XY@1 <-> to_rail_XY@131 [Mate]: SAR340-40_r:1 ↔ SAR3_ba:128
- to_ball4_17_Z@1 <-> to_rail_Z@131 [Mate]: SAR340-40_r:1 ↔ SAR3_ba:128
- to_ball4_17_YZ@1 <-> to_rail_YZ@131 [Angle] (0 deg): SAR340-40_r:1 ↔ SAR3_ba:128
- to_ball4_18_XY@1 <-> to_rail_XY@132 [Mate]: SAR340-40_r:1 ↔ SAR3_ba:129
- to_ball4_18_Z@1 <-> to_rail_Z@132 [Mate]: SAR340-40_r:1 ↔ SAR3_ba:129
- to_ball4_18_YZ@1 <-> to_rail_YZ@132 [Angle] (0 deg): SAR340-40_r:1 ↔ SAR3_ba:129
- to_ball4_19_XY@1 <-> to_rail_XY@133 [Mate]: SAR340-40_r:1 ↔ SAR3_ba:130
- to_ball4_19_Z@1 <-> to_rail_Z@133 [Mate]: SAR340-40_r:1 ↔ SAR3_ba:130
- to_ball4_19_YZ@1 <-> to_rail_YZ@133 [Angle] (0 deg): SAR340-40_r:1 ↔ SAR3_ba:130
- to_ball4_20_XY@1 <-> to_rail_XY@134 [Mate]: SAR340-40_r:1 ↔ SAR3_ba:131
- to_ball4_20_Z@1 <-> to_rail_Z@134 [Mate]: SAR340-40_r:1 ↔ SAR3_ba:131
- to_ball4_20_YZ@1 <-> to_rail_YZ@134 [Angle] (0 deg): SAR340-40_r:1 ↔ SAR3_ba:131
- to_ball4_21_XY@1 <-> to_rail_XY@135 [Mate]: SAR340-40_r:1 ↔ SAR3_ba:132
- to_ball4_21_Z@1 <-> to_rail_Z@135 [Mate]: SAR340-40_r:1 ↔ SAR3_ba:132
- to_ball4_21_YZ@1 <-> to_rail_YZ@135 [Angle] (0 deg): SAR340-40_r:1 ↔ SAR3_ba:132
- to_ball4_22_XY@1 <-> to_rail_XY@136 [Mate]: SAR340-40_r:1 ↔ SAR3_ba:133
- to_ball4_22_Z@1 <-> to_rail_Z@136 [Mate]: SAR340-40_r:1 ↔ SAR3_ba:133
- to_ball4_22_YZ@1 <-> to_rail_YZ@136 [Angle] (0 deg): SAR340-40_r:1 ↔ SAR3_ba:133
- to_ball4_23_XY@1 <-> to_rail_XY@137 [Mate]: SAR340-40_r:1 ↔ SAR3_ba:134
- to_ball4_23_Z@1 <-> to_rail_Z@137 [Mate]: SAR340-40_r:1 ↔ SAR3_ba:134
- to_ball4_23_YZ@1 <-> to_rail_YZ@137 [Angle] (0 deg): SAR340-40_r:1 ↔ SAR3_ba:134
- to_ball4_24_XY@1 <-> to_rail_XY@138 [Mate]: SAR340-40_r:1 ↔ SAR3_ba:135
- to_ball4_24_Z@1 <-> to_rail_Z@138 [Mate]: SAR340-40_r:1 ↔ SAR3_ba:135
- to_ball4_24_YZ@1 <-> to_rail_YZ@138 [Angle] (0 deg): SAR340-40_r:1 ↔ SAR3_ba:135
- to_ball4_25_XY@1 <-> to_rail_XY@139 [Mate]: SAR340-40_r:1 ↔ SAR3_ba:136
- to_ball4_25_Z@1 <-> to_rail_Z@139 [Mate]: SAR340-40_r:1 ↔ SAR3_ba:136
- to_ball4_25_YZ@1 <-> to_rail_YZ@139 [Angle] (0 deg): SAR340-40_r:1 ↔ SAR3_ba:136
- to_ball4_26_XY@1 <-> to_rail_XY@140 [Mate]: SAR340-40_r:1 ↔ SAR3_ba:137
- to_ball4_26_Z@1 <-> to_rail_Z@140 [Mate]: SAR340-40_r:1 ↔ SAR3_ba:137
- to_ball4_26_YZ@1 <-> to_rail_YZ@140 [Angle] (0 deg): SAR340-40_r:1 ↔ SAR3_ba:137
- to_ball4_27_XY@1 <-> to_rail_XY@141 [Mate]: SAR340-40_r:1 ↔ SAR3_ba:138
- to_ball4_27_Z@1 <-> to_rail_Z@141 [Mate]: SAR340-40_r:1 ↔ SAR3_ba:138
- to_ball4_27_YZ@1 <-> to_rail_YZ@141 [Angle] (0 deg): SAR340-40_r:1 ↔ SAR3_ba:138
- to_ball4_28_XY@1 <-> to_rail_XY@142 [Mate]: SAR340-40_r:1 ↔ SAR3_ba:139
- to_ball4_28_Z@1 <-> to_rail_Z@142 [Mate]: SAR340-40_r:1 ↔ SAR3_ba:139
- to_ball4_28_YZ@1 <-> to_rail_YZ@142 [Angle] (0 deg): SAR340-40_r:1 ↔ SAR3_ba:139
- to_ball4_29_XY@1 <-> to_rail_XY@143 [Mate]: SAR340-40_r:1 ↔ SAR3_ba:140
- to_ball4_29_Z@1 <-> to_rail_Z@143 [Mate]: SAR340-40_r:1 ↔ SAR3_ba:140
- to_ball4_29_YZ@1 <-> to_rail_YZ@143 [Angle] (0 deg): SAR340-40_r:1 ↔ SAR3_ba:140
- to_ball4_30_XY@1 <-> to_rail_XY@144 [Mate]: SAR340-40_r:1 ↔ SAR3_ba:141
- to_ball4_30_Z@1 <-> to_rail_Z@144 [Mate]: SAR340-40_r:1 ↔ SAR3_ba:141
- to_ball4_30_YZ@1 <-> to_rail_YZ@144 [Angle] (0 deg): SAR340-40_r:1 ↔ SAR3_ba:141
- to_ball4_31_XY@1 <-> to_rail_XY@145 [Mate]: SAR340-40_r:1 ↔ SAR3_ba:142
- to_ball4_31_Z@1 <-> to_rail_Z@145 [Mate]: SAR340-40_r:1 ↔ SAR3_ba:142
- to_ball4_31_YZ@1 <-> to_rail_YZ@145 [Angle] (0 deg): SAR340-40_r:1 ↔ SAR3_ba:142
- to_ball4_32_XY@1 <-> to_rail_XY@146 [Mate]: SAR340-40_r:1 ↔ SAR3_ba:143
- to_ball4_32_Z@1 <-> to_rail_Z@146 [Mate]: SAR340-40_r:1 ↔ SAR3_ba:143
- to_ball4_32_YZ@1 <-> to_rail_YZ@146 [Angle] (0 deg): SAR340-40_r:1 ↔ SAR3_ba:143
- to_ball4_33_XY@1 <-> to_rail_XY@147 [Mate]: SAR340-40_r:1 ↔ SAR3_ba:144
- to_ball4_33_Z@1 <-> to_rail_Z@147 [Mate]: SAR340-40_r:1 ↔ SAR3_ba:144
- to_ball4_33_YZ@1 <-> to_rail_YZ@147 [Angle] (0 deg): SAR340-40_r:1 ↔ SAR3_ba:144
- to_ball4_34_XY@1 <-> to_rail_XY@148 [Mate]: SAR340-40_r:1 ↔ SAR3_ba:145
- to_ball4_34_Z@1 <-> to_rail_Z@148 [Mate]: SAR340-40_r:1 ↔ SAR3_ba:145
- to_ball4_34_YZ@1 <-> to_rail_YZ@148 [Angle] (0 deg): SAR340-40_r:1 ↔ SAR3_ba:145
- to_ball4_35_XY@1 <-> to_rail_XY@149 [Mate]: SAR340-40_r:1 ↔ SAR3_ba:146
- to_ball4_35_Z@1 <-> to_rail_Z@149 [Mate]: SAR340-40_r:1 ↔ SAR3_ba:146
- to_ball4_35_YZ@1 <-> to_rail_YZ@149 [Angle] (0 deg): SAR340-40_r:1 ↔ SAR3_ba:146
- to_ball4_36_XY@1 <-> to_rail_XY@150 [Mate]: SAR340-40_r:1 ↔ SAR3_ba:147
- to_ball4_36_Z@1 <-> to_rail_Z@150 [Mate]: SAR340-40_r:1 ↔ SAR3_ba:147
- to_ball4_36_YZ@1 <-> to_rail_YZ@150 [Angle] (0 deg): SAR340-40_r:1 ↔ SAR3_ba:147
- to_ball4_37_XY@1 <-> to_rail_XY@151 [Mate]: SAR340-40_r:1 ↔ SAR3_ba:148
- to_ball4_37_Z@1 <-> to_rail_Z@151 [Mate]: SAR340-40_r:1 ↔ SAR3_ba:148
- to_ball4_37_YZ@1 <-> to_rail_YZ@151 [Angle] (0 deg): SAR340-40_r:1 ↔ SAR3_ba:148
- Mate:299: SAR340-40_b:2
- Mate:300: SAR340-40_b:2
- Mate:301: SAR340-40_b:2
- Mate:302: SAR340-40_b:1
- Mate:303: SAR340-40_b:1
- Mate:304: SAR340-40_b:1
- Flush:1 (10 mm): SAR340-40_b:1 ↔ SAR340-40_b:2
